# Autodesk Inventor assembly: Talon with Fan
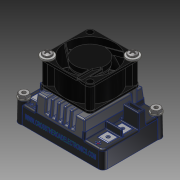
[picture p0: Inventor's stored thumbnail of the model, 180x180]
Saved by Autodesk Inventor 2014 SP1 (Build 180222100, 222)
## iProperties
Created: 2013-01-27
Part Number: Talon with Fan
Document SubType Name: Assembly
Designer: Moses
Mass: 109.125 g
Surface Area: 542.271 cm^2
Volume: 55.3176 cm^3
Density: 1.9727 g/cm^3
Author: Moses
## Documents named in this file (7)
- C:\Users\Moses\Documents\Inventor\Sally Rebuild\Rebuild Sally\Talon with Fan.iam
- C:\Users\Moses\Documents\Inventor\Sally Rebuild\Rebuild Sally\Talon.ipt
- C:\Users\Moses\Documents\Inventor\Sally Rebuild\Rebuild Sally\ELEC_FanMini_412.iam
- C:\Users\Moses\Documents\Inventor\Sally Rebuild\Rebuild Sally\Standard #6 Washer.ipt
- C:\Users\Moses\Documents\Inventor\Sally Rebuild\Rebuild Sally\6-32 18-8 Stainless Steel Pan Head Philips Machine Screw\1.0000\91772A153.ipt
- C:\Users\Moses\Documents\Inventor\Sally Rebuild\Rebuild Sally\Standard #4 Washer.ipt
- C:\Users\Moses\Documents\Inventor\Sally Rebuild\Rebuild Sally\4-40 18-8 Stainless Steel Pan Head Phillips Machine Screw\18-8 Stainless Steel Machine Screw Hex Nut\91841A005.ipt
## Components (10 placed, 6 different names)
1. Talon:1 — Mate:1, Mate:2, Mate:3, Insert:9, Insert:10
2. ELEC_FanMini_412:1 [sub-assembly] — Mate:1, Mate:2, Mate:3, Insert:4, Insert:8
3. Standard #6 Washer:2 — Insert:4
4. 91772A153:2
5. Standard #6 Washer:4 — Insert:8
6. 91772A153:4
7. Standard #4 Washer:1 — Insert:9, Insert:12
8. Standard #4 Washer:2 — Insert:10, Insert:11
9. 91841A005:1 — Insert:12
10. 91841A005:2 — Insert:11
## Relationships (11: Insert 8, Mate 3)
- Mate:1: Talon:1 ↔ ELEC_FanMini_412:1
- Mate:2 (14.4018 mm): Talon:1 ↔ ELEC_FanMini_412:1
- Mate:3 (4.2418 mm): Talon:1 ↔ ELEC_FanMini_412:1
- [Insert]: Standard #6 Washer:2 ↔ 91772A153:2
- Insert:4: ELEC_FanMini_412:1 ↔ Standard #6 Washer:2
- [Insert]: Standard #6 Washer:4 ↔ 91772A153:4
- Insert:8: ELEC_FanMini_412:1 ↔ Standard #6 Washer:4
- Insert:9: Talon:1 ↔ Standard #4 Washer:1
- Insert:10: Talon:1 ↔ Standard #4 Washer:2
- Insert:11: Standard #4 Washer:2 ↔ 91841A005:2
- Insert:12: Standard #4 Washer:1 ↔ 91841A005:1
## Named parameters: d5_d4 = 0 mm, d8_d4 = 0 mm
